# Autodesk Inventor assembly: pistonassembly
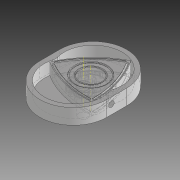
[picture p0: Inventor's stored thumbnail of the model, 180x180]
Saved by Autodesk Inventor 2020 (Build 240168000, 168)
## iProperties
Created: 2020-11-25
Part Number: pistonassembly
Document SubType Name: Assembly
Designer: DDeGo
Author: DDeGo
## Documents named in this file (7)
- C:\Users\DDeGo\Documents\Drew\Projects\AirWankel\cad\pistonassembly.iam
- C:\Users\DDeGo\Documents\Drew\Projects\AirWankel\cad\housing.ipt
- C:\Users\DDeGo\Documents\Drew\Projects\AirWankel\cad\piston.ipt
- C:\Users\DDeGo\Documents\Drew\Projects\AirWankel\cad\camshaft.ipt
- C:\Users\DDeGo\Documents\Drew\Projects\AirWankel\cad\6701 bearing.ipt
- C:\Users\DDeGo\Documents\Drew\Projects\AirWankel\cad\MR85 bearing.ipt
- C:\Users\DDeGo\Documents\Drew\Projects\AirWankel\cad\housingPlate.ipt
## Components (6 placed, 6 different names)
1. housing:1 — Mate:1, Mate:4, Mate:10, Mate:11, Tangent:1, Mate:14
2. piston:1 — Mate:1, Mate:2, Mate:12, Tangent:1
3. camshaft:1 — Mate:4, Mate:5, Mate:8, Mate:13
4. 6701 bearing:1 — Mate:2, Mate:5, Mate:12
5. MR85 bearing:1 — Mate:8, Mate:13, Mate:14
6. housingPlate:1 — Mate:10, Mate:11
## Relationships (11: Mate 10, Tangent 1)
- Mate:1: housing:1 ↔ piston:1
- Mate:2: piston:1 ↔ 6701 bearing:1
- Mate:4: housing:1 ↔ camshaft:1
- Mate:5: camshaft:1 ↔ 6701 bearing:1
- Mate:8: camshaft:1 ↔ MR85 bearing:1
- Mate:10: housing:1 ↔ housingPlate:1
- Mate:11: housing:1 ↔ housingPlate:1
- Mate:12: piston:1 ↔ 6701 bearing:1
- Tangent:1: housing:1 ↔ piston:1
- Mate:13: camshaft:1 ↔ MR85 bearing:1
- Mate:14: housing:1 ↔ MR85 bearing:1
